# Autodesk Inventor assembly: FullAssembly
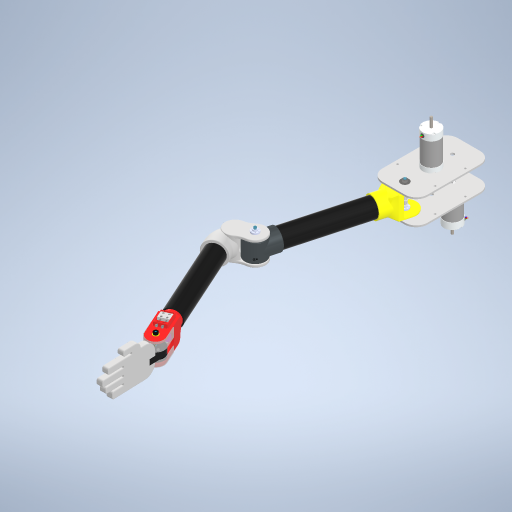
[picture p0: Inventor's stored thumbnail of the model, 512x512]
Saved by Autodesk Inventor 2024 (Build 280153000, 153)
## iProperties
Created: 2024-03-12
Part Number: FullAssembly
Document SubType Name: Assembly
Designer: Irwin
Author: Irwin
## Documents named in this file (17)
- C:\Users\anyangoe\Desktop\WholeRobot\FullAssembly.iam
- C:\Users\anyangoe\Desktop\WholeRobot\Plate.ipt
- C:\Users\anyangoe\Desktop\WholeRobot\ShoulderConnector.ipt
- C:\Users\anyangoe\Desktop\WholeRobot\8mmShaft.ipt
- C:\Users\anyangoe\Desktop\WholeRobot\FlangedBearing.ipt
- C:\Users\anyangoe\Desktop\WholeRobot\8mmShaftCollar.ipt
- C:\Users\anyangoe\Desktop\WholeRobot\mounting-hub-8mm-shaft-m3-holes.ipt
- C:\Users\anyangoe\Desktop\WholeRobot\Spindle Motor.ipt
- C:\Users\anyangoe\Desktop\WholeRobot\GT2 Timing Pulley 20T 10mm - Bore_8mm.iam
- C:\Users\anyangoe\Desktop\WholeRobot\GT2 Timing Pulley 40T 10mm - Bore_8mm.ipt
- C:\Users\anyangoe\Desktop\WholeRobot\GT2 Idler Pulley 20 Tooth 9mm Wide.ipt
- C:\Users\anyangoe\Desktop\WholeRobot\Tube.ipt
- C:\Users\anyangoe\Desktop\WholeRobot\ElbowAssembly.iam
- C:\Users\anyangoe\Desktop\WholeRobot\WristAssembly.iam
- WristAssembly.iam
- C:\Users\anyangoe\Desktop\WholeRobot\wrist-cover-bottom.ipt
- C:\Users\anyangoe\Desktop\WholeRobot\wrist-cover-top.ipt
## Components (22 placed, 15 different names)
1. Plate:1 — Mate:1, Mate:3, Mate:4, Flush:1, Mate:5, Mate:8, Mate:13, Mate:22, Mate:23, Mate:28
2. ShoulderConnector:1 — Mate:1, Mate:5, Mate:6, Mate:7, Mate:9, Mate:19, Mate:32, Mate:33
3. Plate:2 — Mate:6, Mate:7, Mate:8, Flush:2, Mate:12, Mate:20, Mate:21, Mate:25, Angle:1
4. 8mmShaft:1 — Mate:9, Flush:2, Mate:10, Mate:11, Mate:14, Mate:15, Mate:18, Mate:26, Mate:29, Mate:30
5. FlangedBearing:1 — Mate:10, Mate:12, Mate:16
6. FlangedBearing:2 — Mate:11, Mate:13, Mate:17
7. 8mmShaftCollar:1 — Mate:15, Mate:16
8. 8mmShaftCollar:2 — Mate:14, Mate:17
9. mounting-hub-8mm-shaft-m3-holes:1 — Mate:18, Mate:19, To Stop From Moving
10. Spindle Motor:1 — Mate:20, Mate:21, Mate:24
11. Spindle Motor:2 — Mate:22, Mate:23, Mate:27
12. GT2 Timing Pulley 20T 10mm - Bore_8mm:1 [sub-assembly] — Mate:24, Mate:25, Flush:3
13. GT2 Timing Pulley 40T 10mm - Bore_8mm:1 — Mate:26, Flush:3
14. GT2 Timing Pulley 20T 10mm - Bore_8mm:2 [sub-assembly] — Mate:27, Mate:28
15. GT2 Idler Pulley 20 Tooth 9mm Wide:1 — Mate:29, Mate:31, To Stop From Moving
16. GT2 Idler Pulley 20 Tooth 9mm Wide:2 — Mate:30, Mate:31
17. Tube:1 — Mate:32, Mate:33, Mate:34, Mate:38
18. Tube:2 — Mate:35, Mate:36, Mate:37, Mate:39
19. ElbowAssembly:1 [sub-assembly] — Mate:34, Angle:1, Mate:35, Mate:36, Angle:2, Mate:38
20. WristAssembly:1 [sub-assembly] — Mate:37, Angle:2, Mate:39, Mate:40, Angle:3, Flush:4, Mate:41, Angle:4, Flush:5
21. wrist-cover-bottom:1 — Mate:41, Angle:4, Flush:5
22. wrist-cover-top:1 — Mate:40, Angle:3, Flush:4
## Relationships (50: Mate 41, Flush 5, Angle 4)
- Mate:1: Plate:1 ↔ ShoulderConnector:1
- Mate:3: Plate:1
- Mate:4: Plate:1
- Flush:1: Plate:1
- Mate:5: Plate:1 ↔ ShoulderConnector:1
- Mate:6: ShoulderConnector:1 ↔ Plate:2
- Mate:7: ShoulderConnector:1 ↔ Plate:2
- Mate:8: Plate:1 ↔ Plate:2
- Mate:9: ShoulderConnector:1 ↔ 8mmShaft:1
- Flush:2 (-10 mm): Plate:2 ↔ 8mmShaft:1
- Mate:10: 8mmShaft:1 ↔ FlangedBearing:1
- Mate:11: 8mmShaft:1 ↔ FlangedBearing:2
- Mate:12: Plate:2 ↔ FlangedBearing:1
- Mate:13: Plate:1 ↔ FlangedBearing:2
- Mate:14: 8mmShaft:1 ↔ 8mmShaftCollar:2
- Mate:15: 8mmShaft:1 ↔ 8mmShaftCollar:1
- Mate:16: FlangedBearing:1 ↔ 8mmShaftCollar:1
- Mate:17: FlangedBearing:2 ↔ 8mmShaftCollar:2
- Mate:18: 8mmShaft:1 ↔ mounting-hub-8mm-shaft-m3-holes:1
- Mate:19: ShoulderConnector:1 ↔ mounting-hub-8mm-shaft-m3-holes:1
- Mate:20: Plate:2 ↔ Spindle Motor:1
- Mate:21: Plate:2 ↔ Spindle Motor:1
- Mate:22: Plate:1 ↔ Spindle Motor:2
- Mate:23: Plate:1 ↔ Spindle Motor:2
- Mate:24: Spindle Motor:1 ↔ GT2 Timing Pulley 20T 10mm - Bore_8mm:1
- Mate:25: Plate:2 ↔ GT2 Timing Pulley 20T 10mm - Bore_8mm:1
- Mate:26: 8mmShaft:1 ↔ GT2 Timing Pulley 40T 10mm - Bore_8mm:1
- Flush:3: GT2 Timing Pulley 20T 10mm - Bore_8mm:1 ↔ GT2 Timing Pulley 40T 10mm - Bore_8mm:1
- Mate:27: Spindle Motor:2 ↔ GT2 Timing Pulley 20T 10mm - Bore_8mm:2
- Mate:28: Plate:1 ↔ GT2 Timing Pulley 20T 10mm - Bore_8mm:2
- Mate:29: 8mmShaft:1 ↔ GT2 Idler Pulley 20 Tooth 9mm Wide:1
- Mate:30: 8mmShaft:1 ↔ GT2 Idler Pulley 20 Tooth 9mm Wide:2
- Mate:31: GT2 Idler Pulley 20 Tooth 9mm Wide:1 ↔ GT2 Idler Pulley 20 Tooth 9mm Wide:2
- Mate:32: ShoulderConnector:1 ↔ Tube:1
- Mate:33 (-19.05 mm): ShoulderConnector:1 ↔ Tube:1
- Mate:34: Tube:1 ↔ ElbowAssembly:1
- Angle:1 (0 deg): Plate:2 ↔ ElbowAssembly:1
- Mate:35: Tube:2 ↔ ElbowAssembly:1
- Mate:36: Tube:2 ↔ ElbowAssembly:1
- Mate:37: Tube:2 ↔ WristAssembly:1
- Angle:2 (0 deg): ElbowAssembly:1 ↔ WristAssembly:1
- Mate:38: Tube:1 ↔ ElbowAssembly:1
- Mate:39 (-90 mm): Tube:2 ↔ WristAssembly:1
- Mate:40: WristAssembly:1 ↔ wrist-cover-top:1
- Angle:3 (180 deg): WristAssembly:1 ↔ wrist-cover-top:1
- Flush:4: WristAssembly:1 ↔ wrist-cover-top:1
- Mate:41: WristAssembly:1 ↔ wrist-cover-bottom:1
- Angle:4 (0 deg): WristAssembly:1 ↔ wrist-cover-bottom:1
- Flush:5: WristAssembly:1 ↔ wrist-cover-bottom:1
- To Stop From Moving [Mate] (2 mm): mounting-hub-8mm-shaft-m3-holes:1 ↔ GT2 Idler Pulley 20 Tooth 9mm Wide:1
